# Autodesk Inventor assembly: Motot_Gear_Enclosure_Assembly
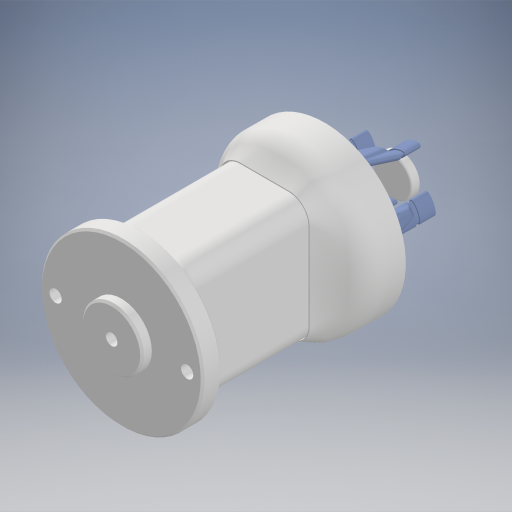
[picture p0: Inventor's stored thumbnail of the model, 512x512]
Saved by Autodesk Inventor 2024 (Build 280153000, 153)
## iProperties
Created: 2024-03-16
Part Number: Motot_Gear_Enclosure_Assembly
Document SubType Name: Assembly
Designer: Faber
Author: Faber
## Documents named in this file (6)
- C:\Users\Bluex\OneDrive - Syddansk Universitet\2. Semester\Autonome_Robotter\Gripper_3D-Files\Motot_Gear_Enclosure_Assembly.iam
- C:\Users\Bluex\OneDrive - Syddansk Universitet\2. Semester\Autonome_Robotter\Gripper_3D-Files\Motor_in_Enclosure.iam
- C:\Users\Bluex\OneDrive - Syddansk Universitet\2. Semester\Autonome_Robotter\Gripper_3D-Files\Gear_Enclosure.ipt
- C:\Users\Bluex\OneDrive - Syddansk Universitet\2. Semester\Autonome_Robotter\Gripper_3D-Files\Gear_Assembly\Design Accelerator\Spur Gear11.ipt
- C:\Users\Bluex\OneDrive - Syddansk Universitet\2. Semester\Autonome_Robotter\Gripper_3D-Files\Gear_Assembly\Design Accelerator\Spur Gear21.ipt
- C:\Users\Bluex\OneDrive - Syddansk Universitet\2. Semester\Autonome_Robotter\Gripper_3D-Files\Brikker.ipt
## Components (8 placed, 5 different names)
1. Motor_in_Enclosure:1 [sub-assembly] — Mate:1, Mate:2, Mate:3, Mate:4, Mate:13
2. Gear_Enclosure:1 — Mate:1, Mate:2, Mate:3, Mate:5, Mate:6, Mate:7, Mate:8, Mate:9, Mate:10, Mate:11, Mate:12
3. Spur Gear1:1 — Mate:13, Flush:1, Rotation:1, Rotation:2, Rotation:3, Rotation:4
4. Spur Gear2:1 — Mate:11, Mate:12, Flush:1, Rotation:2
5. Spur Gear2:2 — Mate:5, Mate:6, Rotation:4
6. Spur Gear2:3 — Mate:9, Mate:10, Rotation:3, Flush:2
7. Spur Gear2:4 — Mate:7, Mate:8, Rotation:1
8. Brikker:1 — Flush:2
## Relationships (19: Mate 13, RelateRotation 4, Flush 2)
- Mate:1: Motor_in_Enclosure:1 ↔ Gear_Enclosure:1
- Mate:2: Motor_in_Enclosure:1 ↔ Gear_Enclosure:1
- Mate:3: Motor_in_Enclosure:1 ↔ Gear_Enclosure:1
- Mate:4: Motor_in_Enclosure:1
- Mate:5: Gear_Enclosure:1 ↔ Spur Gear2:2
- Mate:6: Gear_Enclosure:1 ↔ Spur Gear2:2
- Mate:7: Gear_Enclosure:1 ↔ Spur Gear2:4
- Mate:8: Gear_Enclosure:1 ↔ Spur Gear2:4
- Mate:9: Gear_Enclosure:1 ↔ Spur Gear2:3
- Mate:10: Gear_Enclosure:1 ↔ Spur Gear2:3
- Mate:11: Gear_Enclosure:1 ↔ Spur Gear2:1
- Mate:12: Gear_Enclosure:1 ↔ Spur Gear2:1
- Mate:13: Motor_in_Enclosure:1 ↔ Spur Gear1:1
- Flush:1: Spur Gear1:1 ↔ Spur Gear2:1
- Rotation:1 [RelateRotation] (0.5714 ul): Spur Gear1:1 ↔ Spur Gear2:4
- Rotation:2 [RelateRotation] (0.5714 ul): Spur Gear1:1 ↔ Spur Gear2:1
- Rotation:3 [RelateRotation] (0.5714 ul): Spur Gear1:1 ↔ Spur Gear2:3
- Rotation:4 [RelateRotation] (0.5714 ul): Spur Gear1:1 ↔ Spur Gear2:2
- Flush:2: Spur Gear2:3 ↔ Brikker:1
